# Autodesk Inventor assembly: Botty
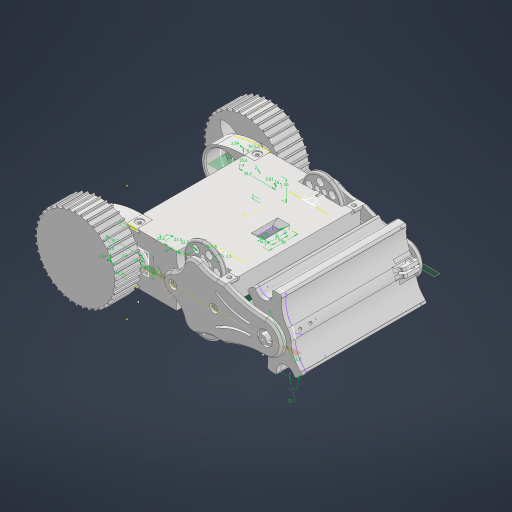
[picture p0: Inventor's stored thumbnail of the model, 512x512]
Saved by Autodesk Inventor 2024.2 (Build 282272000, 272)
## iProperties
Created: 2024-04-12
Part Number: Botty
Document SubType Name: Assembly
Designer: jerem
Author: jerem
## Documents named in this file (9)
- C:\Users\jerem\Documents\GitHub\BOTTY\Botty.iam
- C:\Users\jerem\Documents\GitHub\BOTTY\Body.ipt
- C:\Users\jerem\Documents\GitHub\BOTTY\Body_Cover.ipt
- C:\Users\jerem\Documents\GitHub\BOTTY\BLDC_Arm.ipt
- C:\Users\jerem\Documents\GitHub\BOTTY\Bearing_Arm.ipt
- C:\Users\jerem\Documents\GitHub\BOTTY\Support_Wheel.ipt
- C:\Users\jerem\Documents\GitHub\BOTTY\Drive_Wheel_Bracket.ipt
- C:\Users\jerem\Documents\GitHub\BOTTY\Drive_Wheel.ipt
- C:\Users\jerem\Documents\GitHub\BOTTY\Drum.ipt
## Components (13 placed, 8 different names)
1. Body:1 — Mate:1, Mate:2, Mate:3, Mate:4, Flush:1, Mate:5, Mate:6, Mate:7, Mate:8, Mate:17, Flush:2, Mate:18, Mate:19, Mate:20, Mate:21
2. Body_Cover:1 — Mate:1, Mate:2, Mate:3
3. BLDC_Arm:1 — Mate:4, Flush:1, Mate:5, Mate:13, Mate:14, Mate:15, Mate:16, Mate:28
4. Bearing_Arm:1 — Mate:6, Mate:7, Mate:8, Mate:9, Mate:10, Mate:11, Mate:12, Mate:27
5. Support_Wheel:1 — Mate:15, Mate:16
6. Support_Wheel:2 — Mate:11, Mate:12
7. Support_Wheel:3 — Mate:13, Mate:14
8. Support_Wheel:4 — Mate:9, Mate:10
9. Drive_Wheel_Bracket:1 — Mate:18, Mate:19, Mate:21, Mate:25, Mate:26
10. Drive_Wheel_Bracket:2 — Mate:17, Flush:2, Mate:20, Mate:23, Mate:24
11. Drive_Wheel:1 — Mate:23, Mate:24
12. Drive_Wheel:2 — Mate:25, Mate:26
13. Drum:1 — Mate:27, Mate:28
## Relationships (29: Mate 27, Flush 2)
- Mate:1: Body:1 ↔ Body_Cover:1
- Mate:2: Body:1 ↔ Body_Cover:1
- Mate:3: Body:1 ↔ Body_Cover:1
- Mate:4: Body:1 ↔ BLDC_Arm:1
- Flush:1: Body:1 ↔ BLDC_Arm:1
- Mate:5: Body:1 ↔ BLDC_Arm:1
- Mate:6: Body:1 ↔ Bearing_Arm:1
- Mate:7: Body:1 ↔ Bearing_Arm:1
- Mate:8: Body:1 ↔ Bearing_Arm:1
- Mate:9: Bearing_Arm:1 ↔ Support_Wheel:4
- Mate:10: Bearing_Arm:1 ↔ Support_Wheel:4
- Mate:11: Bearing_Arm:1 ↔ Support_Wheel:2
- Mate:12: Bearing_Arm:1 ↔ Support_Wheel:2
- Mate:13: BLDC_Arm:1 ↔ Support_Wheel:3
- Mate:14: BLDC_Arm:1 ↔ Support_Wheel:3
- Mate:15: BLDC_Arm:1 ↔ Support_Wheel:1
- Mate:16: BLDC_Arm:1 ↔ Support_Wheel:1
- Mate:17: Body:1 ↔ Drive_Wheel_Bracket:2
- Flush:2: Body:1 ↔ Drive_Wheel_Bracket:2
- Mate:18: Body:1 ↔ Drive_Wheel_Bracket:1
- Mate:19: Body:1 ↔ Drive_Wheel_Bracket:1
- Mate:20: Body:1 ↔ Drive_Wheel_Bracket:2
- Mate:21: Body:1 ↔ Drive_Wheel_Bracket:1
- Mate:23: Drive_Wheel_Bracket:2 ↔ Drive_Wheel:1
- Mate:24: Drive_Wheel_Bracket:2 ↔ Drive_Wheel:1
- Mate:25: Drive_Wheel_Bracket:1 ↔ Drive_Wheel:2
- Mate:26: Drive_Wheel_Bracket:1 ↔ Drive_Wheel:2
- Mate:27: Bearing_Arm:1 ↔ Drum:1
- Mate:28 (3.4 mm): BLDC_Arm:1 ↔ Drum:1
